# Autodesk Inventor assembly: main
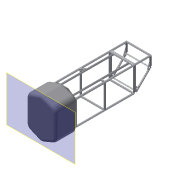
[picture p0: Inventor's stored thumbnail of the model, 180x180]
Saved by Autodesk Inventor 2014 SP1 (Build 180222100, 222)
## iProperties
Created: 2015-02-04
Part Number: main
Document SubType Name: Assembly
Designer: Simen
Author: Simen
## Documents named in this file (5)
- C:\Users\Simen\Documents\git\Eit\skjellet\main.iam
- C:\Users\Simen\Documents\git\Eit\skjellet\base.iam
- C:\Users\Simen\Documents\git\Eit\skjellet\skellett.iam
- C:\Users\Simen\Documents\git\Eit\skjellet\Head.iam
- C:\Users\Simen\Documents\git\Eit\skjellet\HBLFSN5.iam
## Components (4 placed, 4 different names)
1. base:1 [sub-assembly] — Mate:5, Flush:16, Flush:17, Mate:7, Mate:8
2. skellett:1 [sub-assembly] — Mate:5, Flush:16, Flush:17, Mate:6, Flush:18, Flush:19
3. Head:1 [sub-assembly] — Mate:6, Flush:18, Flush:19, Flush:20, Mate:9, Mate:10
4. HBLFSN5:1 [sub-assembly] — Flush:20, Mate:9, Mate:10
## Relationships (11: Mate 6, Flush 5)
- Mate:5: base:1 ↔ skellett:1
- Flush:16 (6 mm): base:1 ↔ skellett:1
- Flush:17 (92 mm): base:1 ↔ skellett:1
- Mate:6: skellett:1 ↔ Head:1
- Mate:7: base:1
- Mate:8: base:1
- Flush:18: skellett:1 ↔ Head:1
- Flush:19: skellett:1 ↔ Head:1
- Flush:20: Head:1 ↔ HBLFSN5:1
- Mate:9: Head:1 ↔ HBLFSN5:1
- Mate:10: Head:1 ↔ HBLFSN5:1
